# Autodesk Inventor assembly: esp32-box-test
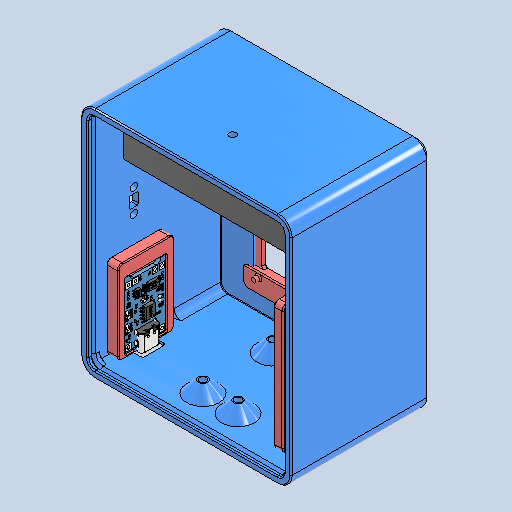
[picture p0: Inventor's stored thumbnail of the model, 512x512]
Saved by Autodesk Inventor 2026 (Build 300175050, 175E)
## iProperties
Created: 2025-06-21
Part Number: esp32-box-test
Document SubType Name: Assembly
Designer: queezz
Author: queezz
## Documents named in this file (8)
- C:\Users\queez\Dropbox\Drawings\PIHTI\ElectronicsBox\esp32-ambient-logger\esp32-box-test.iam
- C:\Users\queez\Dropbox\Drawings\PIHTI\ElectronicsBox\esp32-ambient-logger\esp32-oled-box.iam
- C:\Users\queez\Dropbox\Drawings\PIHTI\ElectronicsBox\esp32-ambient-logger\box-test.ipt
- C:\Users\queez\Dropbox\Drawings\PIHTI\ElectronicsBox\esp32-ambient-logger\STEPs\ESP32-DevkitC32U\ESP32-DevkitC32U.iam
- C:\Users\queez\Dropbox\Drawings\PIHTI\ElectronicsBox\esp32-ambient-logger\esp32-holeless-clip.ipt
- C:\Users\queez\Dropbox\Drawings\PIHTI\ElectronicsBox\esp32-ambient-logger\STEPs\TP4056_Charging_Module_Type_C.iam
- C:\Users\queez\Dropbox\Drawings\PIHTI\ElectronicsBox\esp32-ambient-logger\tp4056-pad.ipt
- C:\Users\queez\Dropbox\Drawings\PIHTI\ElectronicsBox\esp32-ambient-logger\battery-holder.ipt
## Components (7 placed, 7 different names)
1. esp32-oled-box:1 [sub-assembly] — Mate:4, Flush:2, Mate:5
2. box-test:1 — Mate:4, Flush:2, Mate:5, Mate:9, Flush:3, Mate:10, Mate:11, Rotational:1
3. ESP32-DevkitC32U:1 [sub-assembly] — Flush:1, Mate:1, Mate:2
4. esp32-holeless-clip:1 — Flush:1, Mate:1, Mate:2, Rotational:1
5. TP4056_Charging_Module_Type_C:1 [sub-assembly] — Mate:6, Mate:7, Mate:8
6. tp4056-pad:1 — Mate:6, Mate:7, Mate:8, Mate:9, Flush:3, Mate:10
7. battery-holder:1 — Mate:11
## Relationships (14: Mate 10, Flush 3, RevoluteJoint 1)
- Flush:1: ESP32-DevkitC32U:1 ↔ esp32-holeless-clip:1
- Mate:1: ESP32-DevkitC32U:1 ↔ esp32-holeless-clip:1
- Mate:2: ESP32-DevkitC32U:1 ↔ esp32-holeless-clip:1
- Mate:4: esp32-oled-box:1 ↔ box-test:1
- Flush:2: esp32-oled-box:1 ↔ box-test:1
- Mate:5 (-4 mm): esp32-oled-box:1 ↔ box-test:1
- Mate:6: TP4056_Charging_Module_Type_C:1 ↔ tp4056-pad:1
- Mate:7: TP4056_Charging_Module_Type_C:1 ↔ tp4056-pad:1
- Mate:8: TP4056_Charging_Module_Type_C:1 ↔ tp4056-pad:1
- Mate:9: box-test:1 ↔ tp4056-pad:1
- Flush:3 (8 mm): box-test:1 ↔ tp4056-pad:1
- Mate:10: box-test:1 ↔ tp4056-pad:1
- Mate:11: box-test:1 ↔ battery-holder:1
- Rotational:1 [RevoluteJoint]: box-test:1 ↔ esp32-holeless-clip:1
